# Autodesk Inventor assembly: leg_flame_assy
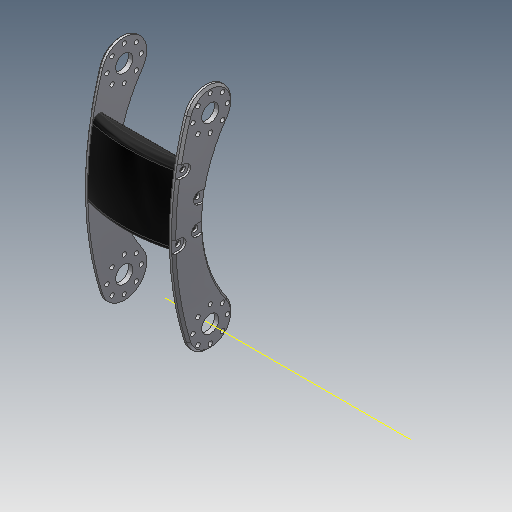
[picture p0: Inventor's stored thumbnail of the model, 512x512]
Saved by Autodesk Inventor 2019.4 (Build 234330000, 330)
## iProperties
Created: 2018-08-12
Part Number: leg_flame_assy
Material: 一般
Document SubType Name: Assembly
Designer: y6tada
Author: y6tada
## Documents named in this file (4)
- C:\Workspace\Yunit8-HaptHexa\Hardware\Inventor\Femur\_Femur.iam
- C:\Workspace\Yunit8-HaptHexa\Hardware\Inventor\Femur\spacer.ipt
- C:\Workspace\Yunit8-HaptHexa\Hardware\Inventor\Femur\side_frame.ipt
- C:\Workspace\Yunit8-HaptHexa\Hardware\Inventor\Femur\side_frame_mir.ipt
## Components (3 placed, 3 different names)
1. leg_spacer — メイト:1, フラッシュ:1, フラッシュ:3, フラッシュ:4
2. side_frame:1 — メイト:1, メイト:6, フラッシュ:2, フラッシュ:3, フラッシュ:4
3. side_frame_mir:1
## Relationships (8: Flush 4, Mate 3, Angle 1)
- メイト:1 [Mate]: leg_spacer ↔ side_frame:1
- メイト:5 [Mate]
- 角度:1 [Angle] (0 deg)
- メイト:6 [Mate]: side_frame:1
- フラッシュ:1 [Flush]: leg_spacer
- フラッシュ:2 [Flush]: side_frame:1
- フラッシュ:3 [Flush]: leg_spacer ↔ side_frame:1
- フラッシュ:4 [Flush]: leg_spacer ↔ side_frame:1
